# Autodesk Inventor assembly: 2AM-17-A-1200 - slider
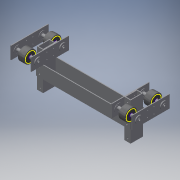
[picture p0: Inventor's stored thumbnail of the model, 180x180]
Saved by Autodesk Inventor 2017 (Build 210142000, 142)
## iProperties
Created: 2017-12-27
Part Number: 2AM-17-A-1200 - slider
Document SubType Name: Assembly
Designer: Micah
Author: Micah
## Documents named in this file (4)
- C:\Users\Micah\Desktop\inventor\CADathon-2017\2AM-17-A-0200 - Smokestack Elevator\2AM-17-A-1200 - moving part.iam
- C:\Users\Micah\Desktop\inventor\CADathon-2017\2AM-17-A-0200 - Smokestack Elevator\2AM-17-P-0203 - moving support.ipt
- C:\Users\Micah\Desktop\inventor\CADathon-2017\2AM-17-A-0200 - Smokestack Elevator\2AM-17-P-0205 - moving structure.ipt
- C:\Users\Micah\Desktop\inventor\CADathon-2017\2AM-17-A-0200 - Smokestack Elevator\2AM-17-A-2200 - slider outside.iam
## Components (6 placed, 3 different names)
1. 2AM-17-P-0203 - moving support:1 — Mate:2, Mate:3
2. 2AM-17-P-0203 - moving support:2
3. 2AM-17-P-0205 - moving structure:2 — Mate:2, Mate:5
4. 2AM-17-A-2200 - slider outside:1 [sub-assembly] — Mate:4
5. 2AM-17-P-0205 - moving structure:3 — Mate:3, Mate:4
6. 2AM-17-A-2200 - slider outside:2 [sub-assembly] — Mate:5
## Relationships (4: Mate 4)
- Mate:2: 2AM-17-P-0203 - moving support:1 ↔ 2AM-17-P-0205 - moving structure:2
- Mate:3: 2AM-17-P-0203 - moving support:1 ↔ 2AM-17-P-0205 - moving structure:3
- Mate:4: 2AM-17-A-2200 - slider outside:1 ↔ 2AM-17-P-0205 - moving structure:3
- Mate:5: 2AM-17-P-0205 - moving structure:2 ↔ 2AM-17-A-2200 - slider outside:2
